# Autodesk Inventor assembly: Montiert
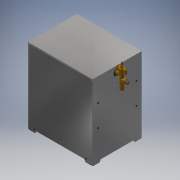
[picture p0: Inventor's stored thumbnail of the model, 180x180]
Saved by Autodesk Inventor 2018 (Build 220112000, 112)
## iProperties
Created: 2017-11-12
Part Number: Montiert
Material: Generisch
Document SubType Name: Assembly
Mass: 12109.4 g
Surface Area: 4943.53 cm^2
Volume: 1535.77 cm^3
Density: 7.8849 g/cm^3
## Documents named in this file (15)
- C:\git\RoKu-ProjectX01\Konstruktion\Montiert.iam
- C:\git\RoKu-ProjectX01\Konstruktion\Brenner.ipt
- C:\git\RoKu-ProjectX01\Konstruktion\BrennerHalter.ipt
- C:\git\RoKu-ProjectX01\Konstruktion\Gegenhalter.ipt
- C:\Users\kuckal\Documents\Inventor\Content Center Files\R2018\de-DE\ISO 7380-1\ISO 7380-1 - M4 x 6.ipt
- C:\Users\kuckal\Documents\Inventor\Content Center Files\R2018\de-DE\ISO 7380-1\ISO 7380-1 - M4 x 8.ipt
- C:\Users\kuckal\Documents\Inventor\Content Center Files\R2018\de-DE\ISO 4036(1)\ISO 4036 - M4(1).ipt
- C:\git\RoKu-ProjectX01\Konstruktion\Front.ipt
- C:\git\RoKu-ProjectX01\Konstruktion\MutterMitUScheibe.ipt
- C:\git\RoKu-ProjectX01\Konstruktion\SeiteRechts.ipt
- C:\git\RoKu-ProjectX01\Konstruktion\SeiteLinks.ipt
- C:\git\RoKu-ProjectX01\Konstruktion\Deckel.ipt
- C:\git\RoKu-ProjectX01\Konstruktion\Boden.ipt
- C:\git\RoKu-ProjectX01\Konstruktion\Back.ipt
- C:\git\RoKu-ProjectX01\Konstruktion\Gasanschluss.ipt
## Components (58 placed, 14 different names)
1. Brenner:1 — Fluchtend:1, Fluchtend:2, Fluchtend:3, Passend:1, Einfügen:1, Einfügen:2, Einfügen:3, Einfügen:4, Einfügen:5, Einfügen:6, Einfügen:7, Einfügen:8, Einfügen:9, Einfügen:10, Einfügen:11, Einfügen:12, Fluchtend:6, Passend:41, Passend:42
2. BrennerHalter:1 — Passend:1, Passend:2, Passend:3, Fluchtend:4, Passend:17, Fluchtend:6, Passend:18, Passend:22
3. Gegenhalter:1 — Passend:3, Passend:4, Einfügen:13, Einfügen:14, Einfügen:15, Einfügen:16, Einfügen:17, Einfügen:18, Einfügen:19, Einfügen:20, Einfügen:21, Einfügen:22, Einfügen:23, Einfügen:24
4. Front:1 — Fluchtend:4, Passend:7, Passend:8, Passend:9, Passend:10, Passend:11, Passend:12, Passend:13, Passend:14, Passend:15, Einfügen:25, Einfügen:26, Einfügen:27, Einfügen:28, Passend:16, Fluchtend:5, Passend:17, Passend:19, Fluchtend:7, Passend:21
5. SeiteRechts:1 — Passend:16, Fluchtend:5, Passend:18, Passend:28, Passend:29, Passend:30, Passend:31, Einfügen:29, Einfügen:30, Fluchtend:9, Fluchtend:10
6. SeiteLinks:1 — Passend:19, Fluchtend:7, Passend:20, Passend:22, Passend:24, Passend:25, Passend:26, Passend:27, Einfügen:31, Einfügen:32
7. Deckel:1 — Passend:20, Passend:21, Passend:23
8. Boden:1 — Fluchtend:8, Passend:32
9. Back:1 — Fluchtend:9, Fluchtend:10, Passend:33, Passend:34, Passend:35, Passend:36, Passend:37, Passend:38, Passend:39, Passend:40, Einfügen:33, Einfügen:34, Einfügen:35, Einfügen:36
10. Gasanschluss:1 — Passend:41, Passend:42, Fluchtend:11
11. ISO 7380-1 M4 x 8:1 — Einfügen:1, Passend:4
12. ISO 7380-1 M4 x 8:2 — Einfügen:2
13. ISO 7380-1 M4 x 8:3 — Einfügen:3
14. ISO 7380-1 M4 x 8:4 — Einfügen:4
15. ISO 7380-1 M4 x 8:5 — Einfügen:5
16. ISO 7380-1 M4 x 8:6 — Einfügen:6
17. ISO 7380-1 M4 x 8:7 — Einfügen:7
18. ISO 7380-1 M4 x 8:8 — Einfügen:8
19. ISO 7380-1 M4 x 8:9 — Einfügen:9
20. ISO 7380-1 M4 x 8:10 — Einfügen:10
21. ISO 7380-1 M4 x 8:11 — Einfügen:11
22. ISO 7380-1 M4 x 8:12 — Einfügen:12
23. DIN EN 24036 M4:1 — Einfügen:13
24. DIN EN 24036 M4:2 — Einfügen:14
25. DIN EN 24036 M4:3 — Einfügen:15
26. DIN EN 24036 M4:4 — Einfügen:16
27. DIN EN 24036 M4:5 — Einfügen:17
28. DIN EN 24036 M4:6 — Einfügen:18
29. DIN EN 24036 M4:7 — Einfügen:19
30. DIN EN 24036 M4:8 — Einfügen:20
31. DIN EN 24036 M4:9 — Einfügen:21
32. DIN EN 24036 M4:10 — Einfügen:22
33. DIN EN 24036 M4:11 — Einfügen:23
34. DIN EN 24036 M4:12 — Einfügen:24
35. MutterMitUScheibe:9 — Passend:37, Passend:38
36. MutterMitUScheibe:10 — Passend:39, Passend:40
37. MutterMitUScheibe:11 — Passend:35, Passend:36
38. MutterMitUScheibe:12 — Passend:33, Passend:34
39. ISO 7380-1 M4 x 6:9 — Einfügen:33
40. ISO 7380-1 M4 x 6:10 — Einfügen:34
41. ISO 7380-1 M4 x 6:11 — Einfügen:35
42. ISO 7380-1 M4 x 6:12 — Einfügen:36
43. MutterMitUScheibe:5 — Passend:24, Passend:25
44. MutterMitUScheibe:6 — Passend:26, Passend:27, Passend:32
45. MutterMitUScheibe:7 — Passend:30, Passend:31
46. MutterMitUScheibe:8 — Passend:28, Passend:29
47. ISO 7380-1 M4 x 6:5 — Einfügen:29
48. ISO 7380-1 M4 x 6:6 — Einfügen:30
49. ISO 7380-1 M4 x 6:7 — Einfügen:31
50. ISO 7380-1 M4 x 6:8 — Einfügen:32
51. MutterMitUScheibe:1 — Passend:9, Passend:14
52. MutterMitUScheibe:2 — Passend:8, Passend:15
53. MutterMitUScheibe:3 — Passend:11, Passend:12
54. MutterMitUScheibe:4 — Passend:10, Passend:13
55. ISO 7380-1 M4 x 6:1 — Einfügen:25
56. ISO 7380-1 M4 x 6:2 — Einfügen:26
57. ISO 7380-1 M4 x 6:3 — Einfügen:27
58. ISO 7380-1 M4 x 6:4 — Einfügen:28
## Relationships (87: Mate 40, Insert 36, Flush 11)
- Fluchtend:1 [Flush]: Brenner:1
- Fluchtend:2 [Flush]: Brenner:1
- Fluchtend:3 [Flush]: Brenner:1
- Passend:1 [Mate]: Brenner:1 ↔ BrennerHalter:1
- Passend:2 [Mate]: BrennerHalter:1
- Passend:3 [Mate]: BrennerHalter:1 ↔ Gegenhalter:1
- Einfügen:1 [Insert]: Brenner:1 ↔ ISO 7380-1 M4 x 8:1
- Einfügen:2 [Insert]: Brenner:1 ↔ ISO 7380-1 M4 x 8:2
- Einfügen:3 [Insert]: Brenner:1 ↔ ISO 7380-1 M4 x 8:3
- Einfügen:4 [Insert]: Brenner:1 ↔ ISO 7380-1 M4 x 8:4
- Einfügen:5 [Insert]: Brenner:1 ↔ ISO 7380-1 M4 x 8:5
- Einfügen:6 [Insert]: Brenner:1 ↔ ISO 7380-1 M4 x 8:6
- Einfügen:7 [Insert]: Brenner:1 ↔ ISO 7380-1 M4 x 8:7
- Einfügen:8 [Insert]: Brenner:1 ↔ ISO 7380-1 M4 x 8:8
- Einfügen:9 [Insert]: Brenner:1 ↔ ISO 7380-1 M4 x 8:9
- Einfügen:10 [Insert]: Brenner:1 ↔ ISO 7380-1 M4 x 8:10
- Einfügen:11 [Insert]: Brenner:1 ↔ ISO 7380-1 M4 x 8:11
- Einfügen:12 [Insert]: Brenner:1 ↔ ISO 7380-1 M4 x 8:12
- Passend:4 [Mate]: Gegenhalter:1 ↔ ISO 7380-1 M4 x 8:1
- Einfügen:13 [Insert]: Gegenhalter:1 ↔ DIN EN 24036 M4:1
- Einfügen:14 [Insert]: Gegenhalter:1 ↔ DIN EN 24036 M4:2
- Einfügen:15 [Insert]: Gegenhalter:1 ↔ DIN EN 24036 M4:3
- Einfügen:16 [Insert]: Gegenhalter:1 ↔ DIN EN 24036 M4:4
- Einfügen:17 [Insert]: Gegenhalter:1 ↔ DIN EN 24036 M4:5
- Einfügen:18 [Insert]: Gegenhalter:1 ↔ DIN EN 24036 M4:6
- Einfügen:19 [Insert]: Gegenhalter:1 ↔ DIN EN 24036 M4:7
- Einfügen:20 [Insert]: Gegenhalter:1 ↔ DIN EN 24036 M4:8
- Einfügen:21 [Insert]: Gegenhalter:1 ↔ DIN EN 24036 M4:9
- Einfügen:22 [Insert]: Gegenhalter:1 ↔ DIN EN 24036 M4:10
- Einfügen:23 [Insert]: Gegenhalter:1 ↔ DIN EN 24036 M4:11
- Einfügen:24 [Insert]: Gegenhalter:1 ↔ DIN EN 24036 M4:12
- Fluchtend:4 [Flush]: BrennerHalter:1 ↔ Front:1
- Passend:7 [Mate]: Front:1
- Passend:8 [Mate]: Front:1 ↔ MutterMitUScheibe:2
- Passend:9 [Mate]: Front:1 ↔ MutterMitUScheibe:1
- Passend:10 [Mate]: Front:1 ↔ MutterMitUScheibe:4
- Passend:11 [Mate]: Front:1 ↔ MutterMitUScheibe:3
- Passend:12 [Mate]: Front:1 ↔ MutterMitUScheibe:3
- Passend:13 [Mate]: Front:1 ↔ MutterMitUScheibe:4
- Passend:14 [Mate]: Front:1 ↔ MutterMitUScheibe:1
- Passend:15 [Mate]: Front:1 ↔ MutterMitUScheibe:2
- Einfügen:25 [Insert]: Front:1 ↔ ISO 7380-1 M4 x 6:1
- Einfügen:26 [Insert]: Front:1 ↔ ISO 7380-1 M4 x 6:2
- Einfügen:27 [Insert]: Front:1 ↔ ISO 7380-1 M4 x 6:3
- Einfügen:28 [Insert]: Front:1 ↔ ISO 7380-1 M4 x 6:4
- Passend:16 [Mate]: Front:1 ↔ SeiteRechts:1
- Fluchtend:5 [Flush]: Front:1 ↔ SeiteRechts:1
- Passend:17 [Mate]: BrennerHalter:1 ↔ Front:1
- Fluchtend:6 [Flush]: Brenner:1 ↔ BrennerHalter:1
- Passend:18 [Mate]: BrennerHalter:1 ↔ SeiteRechts:1
- Passend:19 [Mate]: Front:1 ↔ SeiteLinks:1
- Fluchtend:7 [Flush]: Front:1 ↔ SeiteLinks:1
- Passend:20 [Mate]: SeiteLinks:1 ↔ Deckel:1
- Passend:21 [Mate]: Front:1 ↔ Deckel:1
- Passend:22 [Mate]: BrennerHalter:1 ↔ SeiteLinks:1
- Passend:23 [Mate]: Deckel:1
- Passend:24 [Mate]: SeiteLinks:1 ↔ MutterMitUScheibe:5
- Passend:25 [Mate]: SeiteLinks:1 ↔ MutterMitUScheibe:5
- Passend:26 [Mate]: SeiteLinks:1 ↔ MutterMitUScheibe:6
- Passend:27 [Mate]: SeiteLinks:1 ↔ MutterMitUScheibe:6
- Passend:28 [Mate]: SeiteRechts:1 ↔ MutterMitUScheibe:8
- Passend:29 [Mate]: SeiteRechts:1 ↔ MutterMitUScheibe:8
- Passend:30 [Mate]: SeiteRechts:1 ↔ MutterMitUScheibe:7
- Passend:31 [Mate]: SeiteRechts:1 ↔ MutterMitUScheibe:7
- Einfügen:29 [Insert]: SeiteRechts:1 ↔ ISO 7380-1 M4 x 6:5
- Einfügen:30 [Insert]: SeiteRechts:1 ↔ ISO 7380-1 M4 x 6:6
- Einfügen:31 [Insert]: SeiteLinks:1 ↔ ISO 7380-1 M4 x 6:7
- Einfügen:32 [Insert]: SeiteLinks:1 ↔ ISO 7380-1 M4 x 6:8
- Fluchtend:8 [Flush]: Boden:1
- Passend:32 [Mate]: Boden:1 ↔ MutterMitUScheibe:6
- Fluchtend:9 [Flush]: SeiteRechts:1 ↔ Back:1
- Fluchtend:10 [Flush]: SeiteRechts:1 ↔ Back:1
- Passend:33 [Mate]: Back:1 ↔ MutterMitUScheibe:12
- Passend:34 [Mate]: Back:1 ↔ MutterMitUScheibe:12
- Passend:35 [Mate]: Back:1 ↔ MutterMitUScheibe:11
- Passend:36 [Mate]: Back:1 ↔ MutterMitUScheibe:11
- Passend:37 [Mate]: Back:1 ↔ MutterMitUScheibe:9
- Passend:38 [Mate]: Back:1 ↔ MutterMitUScheibe:9
- Passend:39 [Mate]: Back:1 ↔ MutterMitUScheibe:10
- Passend:40 [Mate]: Back:1 ↔ MutterMitUScheibe:10
- Einfügen:33 [Insert]: Back:1 ↔ ISO 7380-1 M4 x 6:9
- Einfügen:34 [Insert]: Back:1 ↔ ISO 7380-1 M4 x 6:10
- Einfügen:35 [Insert]: Back:1 ↔ ISO 7380-1 M4 x 6:11
- Einfügen:36 [Insert]: Back:1 ↔ ISO 7380-1 M4 x 6:12
- Passend:41 [Mate]: Brenner:1 ↔ Gasanschluss:1
- Passend:42 [Mate]: Brenner:1 ↔ Gasanschluss:1
- Fluchtend:11 [Flush]: Gasanschluss:1
